# Autodesk Inventor assembly: sm_varx
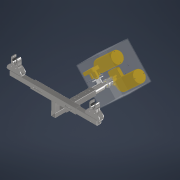
[picture p0: Inventor's stored thumbnail of the model, 180x180]
Saved by Autodesk Inventor 2021 (Build 250183000, 183)
## iProperties
Created: 2021-06-01
Part Number: sm_varx
Document SubType Name: Assembly
Designer: Watchdog
Mass: 2706.84 g
Surface Area: 2512.41 cm^2
Volume: 345.704 cm^3
Density: 7.82995 g/cm^3
Author: Watchdog
## Documents named in this file (15)
- C:\Users\Watchdog\OneDrive - Flinders\Advn Mech Design Shared\6_Development\2_Design\inventor\securing_mechanism\securingMechanism_variant_vertical_x\sm_varx.iam
- C:\Users\Watchdog\OneDrive - Flinders\Advn Mech Design Shared\6_Development\2_Design\inventor\securing_mechanism\securingMechanism_variant_vertical_x\member_axial.ipt
- C:\Users\Watchdog\OneDrive - Flinders\Advn Mech Design Shared\6_Development\2_Design\inventor\securing_mechanism\securingMechanism_variant_vertical_x\member_transverse.ipt
- C:\Users\Watchdog\OneDrive - Flinders\Advn Mech Design Shared\6_Development\2_Design\inventor\securing_mechanism\securingMechanism_variant_vertical_x\member_vertical.ipt
- C:\Users\Watchdog\OneDrive - Flinders\Advn Mech Design Shared\6_Development\2_Design\inventor\securing_mechanism\securingMechanism_variant_vertical_x\member_vertical_inner.ipt
- C:\Users\Watchdog\OneDrive - Flinders\Advn Mech Design Shared\6_Development\2_Design\inventor\securing_mechanism\securingMechanism_variant_vertical_x\member_transverse_inner.ipt
- C:\Users\Watchdog\OneDrive - Flinders\Advn Mech Design Shared\6_Development\2_Design\inventor\securing_mechanism\securingMechanism_variant_vertical_x\assembly_holder3.iam
- C:\Users\Watchdog\OneDrive - Flinders\Advn Mech Design Shared\6_Development\2_Design\inventor\securing_mechanism\connection\sm_connection.iam
- C:\Users\Watchdog\OneDrive - Flinders\Advn Mech Design Shared\6_Development\2_Design\inventor\params.xlsx
- C:\Users\Watchdog\OneDrive - Flinders\Advn Mech Design Shared\6_Development\2_Design\inventor\securing_mechanism\securingMechanism_variant_vertical_x\sm_varx\AIP\FEA\dmzpleppc.fins
- C:\Users\Watchdog\OneDrive - Flinders\Advn Mech Design Shared\6_Development\2_Design\inventor\securing_mechanism\securingMechanism_variant_vertical_x\sm_varx\AIP\FEA\dmzpleppc.fsat
- C:\Users\Watchdog\OneDrive - Flinders\Advn Mech Design Shared\6_Development\2_Design\inventor\securing_mechanism\securingMechanism_variant_vertical_x\sm_varx\AIP\FEA\dmzpleppc.ftes
- C:\Users\Watchdog\OneDrive - Flinders\Advn Mech Design Shared\6_Development\2_Design\inventor\securing_mechanism\securingMechanism_variant_vertical_x\sm_varx\AIP\FEA\dmzpleppc.fwiz
- C:\Users\Watchdog\OneDrive - Flinders\Advn Mech Design Shared\6_Development\2_Design\inventor\securing_mechanism\securingMechanism_variant_vertical_x\sm_varx\AIP\FEA\dmzqhs074.fmsh
- C:\Users\Watchdog\OneDrive - Flinders\Advn Mech Design Shared\6_Development\2_Design\inventor\securing_mechanism\securingMechanism_variant_vertical_x\sm_varx\AIP\FEA\dmzqhs075.fres
## Components (9 placed, 7 different names)
1. member_axial:1 — Mate:2, Flush:5, Mate:10, Flush:13, Flush:14, Flush:15
2. member_transverse:1 — Mate:2, Flush:5, Flush:15, Angle:2, Angle:3, Mate:14, Mate:19
3. member_vertical:1 — Flush:8, Flush:9, Mate:5, Mate:9, Angle:1, Mate:11, Mate:25, Mate:26, Mate:27
4. member_vertical_inner:1 — Mate:9, Angle:1, Mate:10, Flush:13, Flush:14, Mate:11
5. member_transverse_inner:1 — Angle:3, Mate:14, Mate:16, Mate:17, Mate:18
6. member_transverse_inner:2 — Angle:2, Mate:19, Mate:22, Mate:23, Mate:24
7. assembly_holder3:1 [sub-assembly] — Mate:16, Mate:17, Mate:18
8. assembly_holder3:2 [sub-assembly] — Mate:22, Mate:23, Mate:24
9. sm_connection:1 [sub-assembly] — Mate:25, Mate:26, Mate:27
## Relationships (25: Mate 16, Flush 6, Angle 3)
- Mate:2: member_axial:1 ↔ member_transverse:1
- Flush:5 (-2.5 mm): member_axial:1 ↔ member_transverse:1
- Flush:8: member_vertical:1
- Flush:9: member_vertical:1
- Mate:5: member_vertical:1
- Mate:9 (0.5 mm): member_vertical:1 ↔ member_vertical_inner:1
- Angle:1 (0 deg): member_vertical:1 ↔ member_vertical_inner:1
- Mate:10: member_axial:1 ↔ member_vertical_inner:1
- Flush:13: member_axial:1 ↔ member_vertical_inner:1
- Flush:14: member_axial:1 ↔ member_vertical_inner:1
- Mate:11: member_vertical:1 ↔ member_vertical_inner:1
- Flush:15: member_axial:1 ↔ member_transverse:1
- Angle:2 (180 deg): member_transverse:1 ↔ member_transverse_inner:2
- Angle:3 (180 deg): member_transverse:1 ↔ member_transverse_inner:1
- Mate:14 (0.25 mm): member_transverse:1 ↔ member_transverse_inner:1
- Mate:16: member_transverse_inner:1 ↔ assembly_holder3:1
- Mate:17: member_transverse_inner:1 ↔ assembly_holder3:1
- Mate:18: member_transverse_inner:1 ↔ assembly_holder3:1
- Mate:19 (0.25 mm): member_transverse:1 ↔ member_transverse_inner:2
- Mate:22: member_transverse_inner:2 ↔ assembly_holder3:2
- Mate:23: member_transverse_inner:2 ↔ assembly_holder3:2
- Mate:24: member_transverse_inner:2 ↔ assembly_holder3:2
- Mate:25: member_vertical:1 ↔ sm_connection:1
- Mate:26: member_vertical:1 ↔ sm_connection:1
- Mate:27: member_vertical:1 ↔ sm_connection:1
## Named parameters: cover_base_thickness = 10 mm, cover_height_main = 900 mm, cover_length_main = 2200 mm, cover_mountHole_diameter = 10 mm, cover_mountHole_xSpacing = 900 mm, cover_mountHole_ySpacing = 550 mm, cover_shell_thickness = 10 mm, cover_side_openSize = 1400 mm, cover_side_thickness = 20 mm, cover_width_main = 1600 mm, hoop_angle_z = 45 deg, hoop_bearing_length = 5 deg, hoop_cable_diam = 5 mm, hoop_cable_pulley_diam = 22 mm, hoop_height_large = 450 mm, hoop_height_medium = 450 mm, hoop_height_small = 600 mm, hoop_length_large = 200 mm, hoop_length_medium = 700 mm, hoop_length_small = 700 mm, hoop_offset_x = 600 mm, hoop_radius_large = 3300 mm, hoop_thickness_large = 4 mm, hoop_thickness_medium = 3.2 mm, hoop_thickness_small = 2 mm, hoop_width_large = 51 mm, hoop_width_medium = 33.7 mm, hoop_width_small = 25.4 mm, rack_tooth_addendum = 5 mm, rack_tooth_dedendum = 5 mm, rack_tooth_face_widh = 10 mm, rack_tooth_thickness = 5 mm, secure_arm_angle = 35 deg, secure_arm_hold_length = 50 mm, secure_arm_hold_thickness = 30 mm, secure_arm_length = 300 mm, secure_arm_radii = 9 mm, secure_arm_thickness = 30 mm, support_baseClamp_lengthBuffer = 40 mm, support_baseClamp_platformLengthBuffer = 35 mm, support_baseClamp_platformThickness = 15 mm, support_baseClamp_platformWidthBuffer = 0 mm, support_baseClamp_sleeve_hole1Height = 50 mm, support_baseClamp_sleeve_hole2Height = 100 mm, support_baseClamp_sleeveHoleDiameter = 12 mm, support_baseClamp_sleeveSweepTerminationAngle = 55 deg, support_baseClamp_sleeveThickness = 20 mm, support_baseClamp_thickness = 8 mm, support_frame_clampHoleDiameter = 10 mm, support_frame_clampHoleSpacing = 100 mm, support_frame_endHoleBuffer = 25 mm, support_frame_length = 500 mm, support_frame_squareBarDimension = 50 mm, support_frame_squareBarFillet = 2 mm, support_frame_squareBarThickness = 5 mm, testHeight = 1000 mm, testLength = 1700 mm, testWidth = 1500 mm, hoop_tabs_width = 50 mm, hoop_tabs_thickness = 6 mm, hoop_tabs_hole = 12 mm, wheelchair_wheel_radius = 240 mm, wheelchair_deployed_width = 635 mm, wheelchair_deployed_length = 1067 mm, wheelchair_deployed_height = 914 mm, wheelchair_folded_width = 280 mm, sm_varx_squareBarDimension = 30 mm, sm_varx_squareBarThickness = 2.5 mm, sm_varx_x = 50 mm, sm_varx_y = 250 mm, sm_varx_z = 160 mm, sm_varx_pinPlate_thickness = 5 mm, sm_varx_pinPlate_holeDiameter = 5 mm, sm_varx_pinPlate_aspectRatio = 2, sm_varx_member_tolerance = 0.5 mm, a = 2.5 mm, sm_varx_x_arms = 50 mm, hoop_bushing12_radialInterference = 0 mm, hoop_bushing23_radialInterference = 0 mm, hoop_bushing23_od = 27.3 mm, slotDistance = 24 mm, sa_0 = 0, sa_1 = -5632.9, sa_2 = 0, sa_3 = 0, sa_4 = -5632.9, sa_5 = 0, hoop_bushing23_thickness = 1.9 mm, hoop_bushing12_od = 43 mm
note: some values were not read from the file. Shown as the stored number, unit unknown: "sa_0", "sa_1", "sa_2", "sa_3", "sa_4", "sa_5".
